# Autodesk Inventor assembly: Mold Design1
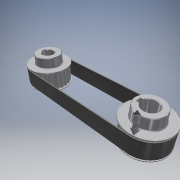
[picture p0: Inventor's stored thumbnail of the model, 180x180]
Saved by Autodesk Inventor 2018 (Build 220112000, 112)
## iProperties
Created: 2018-04-15
Part Number: Mold Design1
Document SubType Name: Assembly
Designer: cwsin_000
Author: cwsin_000
## Documents named in this file (4)
- C:\Users\P241310\Documents\GitHub\mecanum-cad\Mold Design1.iam
- C:\Users\P241310\Documents\GitHub\mecanum-cad\Synchronous Pulley11.ipt
- C:\Users\P241310\Documents\GitHub\mecanum-cad\Synchronous Belt1.ipt
- C:\Users\P241310\Documents\GitHub\mecanum-cad\Synchronous Pulley21.ipt
## Components (3 placed, 3 different names)
1. Synchronous Pulley1:1 — Insert:1
2. Synchronous Belt:1 — Insert:1, Insert:2
3. Synchronous Pulley2:1 — Insert:2
## Relationships (2: Insert 2)
- Insert:1 (-17 mm): Synchronous Pulley1:1 ↔ Synchronous Belt:1
- Insert:2 (-17 mm): Synchronous Belt:1 ↔ Synchronous Pulley2:1
